# Autodesk Inventor assembly: Custom_Delta_Assembly
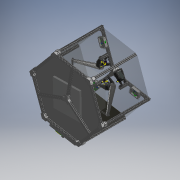
[picture p0: Inventor's stored thumbnail of the model, 180x180]
Saved by Autodesk Inventor 2019.4 (Build 234330000, 330)
## iProperties
Created: 2019-07-06
Part Number: Custom_Delta_Assembly
Document SubType Name: Assembly
Designer: Jorian Brusind
Author: Jorian Brusind
## Documents named in this file (20)
- C:\Users\Jorian Bruslind\Documents\GitHub\ECE44x_Senior_Design\Design files\Delta Robot Arm\Inventor Files\Custom_Delta\Custom_Delta_Assembly.iam
- C:\Users\Jorian Bruslind\Documents\GitHub\ECE44x_Senior_Design\Design files\Delta Robot Arm\Inventor Files\Custom_Delta\Stepper_Face.ipt
- C:\Users\Jorian Bruslind\Documents\GitHub\ECE44x_Senior_Design\Design files\Delta Robot Arm\Inventor Files\Custom_Delta\Delta_Arm.ipt
- C:\Users\Jorian Bruslind\Documents\GitHub\ECE44x_Senior_Design\Design files\Delta Robot Arm\Inventor Files\McMaster Files\5537T518_T-SLOTTED FRAMING.ipt
- C:\Users\Jorian Bruslind\Documents\GitHub\ECE44x_Senior_Design\Design files\Delta Robot Arm\Inventor Files\Custom_Delta\NEMA17_Stepper_CL42H60.ipt
- C:\Users\Jorian Bruslind\Documents\GitHub\ECE44x_Senior_Design\Design files\Delta Robot Arm\Inventor Files\Stepper_Collar\products\12196\step\model.ipt
- C:\Users\Jorian Bruslind\Documents\GitHub\ECE44x_Senior_Design\Design files\Delta Robot Arm\Inventor Files\Custom_Delta\Workarea.ipt
- C:\Users\Jorian Bruslind\Documents\GitHub\ECE44x_Senior_Design\Design files\Delta Robot Arm\Inventor Files\Custom_Delta\Frame_Skeleton.iam
- C:\Users\Jorian Bruslind\Documents\GitHub\ECE44x_Senior_Design\Design files\Delta Robot Arm\Inventor Files\Custom_Delta\350mm_2020_tslot.ipt
- C:\Users\Jorian Bruslind\Documents\GitHub\ECE44x_Senior_Design\Design files\Delta Robot Arm\Inventor Files\Custom_Delta\80_20_top_connector.ipt
- C:\Users\Jorian Bruslind\Documents\GitHub\ECE44x_Senior_Design\Design files\Delta Robot Arm\Inventor Files\McMaster Files\98861A050_LOW-STRENGTH STEEL THREADED ROD.ipt
- C:\Users\Jorian Bruslind\Documents\GitHub\ECE44x_Senior_Design\Design files\Delta Robot Arm\Inventor Files\McMaster Files\59935K140_METRIC BALL JOINT ROD END.ipt
- C:\Users\Jorian Bruslind\Documents\GitHub\ECE44x_Senior_Design\Design files\Delta Robot Arm\Inventor Files\Custom_Delta\End_Effector.iam
- C:\Users\Jorian Bruslind\Documents\GitHub\ECE44x_Senior_Design\Design files\Delta Robot Arm\Inventor Files\Custom_Delta\77mm_2020_tslot.ipt
- C:\Users\Jorian Bruslind\Documents\GitHub\ECE44x_Senior_Design\Design files\Delta Robot Arm\Inventor Files\Custom_Delta\275mm_2020_tslot.ipt
- C:\Users\Jorian Bruslind\Documents\GitHub\ECE44x_Senior_Design\Design files\Delta Robot Arm\Inventor Files\Custom_Delta\Acrylic_bottom.ipt
- C:\Users\Jorian Bruslind\Documents\GitHub\ECE44x_Senior_Design\Design files\Delta Robot Arm\Inventor Files\Custom_Delta\Motor_Node.iam
- C:\Users\Jorian Bruslind\Documents\GitHub\ECE44x_Senior_Design\Design files\Delta Robot Arm\Inventor Files\Custom_Delta\Power_Supply.ipt
- C:\Users\Jorian Bruslind\Documents\GitHub\ECE44x_Senior_Design\Design files\Delta Robot Arm\Inventor Files\Raspberry PI 3\Raspberry Pi 3.iam
- C:\Users\Jorian Bruslind\Documents\GitHub\ECE44x_Senior_Design\Design files\Delta Robot Arm\Inventor Files\Custom_Delta\Acrylic_angle_bracket.ipt
## Components (56 placed, 19 different names)
1. Stepper_Face:1 — Mate:210, Mate:211, Mate:212, Mate:216, Mate:493, Flush:5, Flush:9, Mate:506, Mate:555
2. Delta_Arm:1 — Mate:214, Mate:215, Mate:254, Mate:517, Mate:518, Mate:519, Mate:520
3. Stepper_Face:2 — Mate:222, Mate:227, Mate:230, Mate:231, Mate:491, Flush:10, Mate:505, Mate:553
4. Delta_Arm:2 — Mate:220, Mate:221, Mate:253, Mate:513, Mate:514, Mate:515, Mate:516
5. Stepper_Face:3 — Mate:217, Mate:218, Mate:226, Mate:228, Mate:495, Flush:8, Mate:507, Mate:557
6. Delta_Arm:3 — Mate:224, Mate:225, Mate:229, Mate:509, Mate:510, Mate:511, Mate:512
7. NEMA17_Stepper_CL42H60:1 — Mate:219, Mate:227, Mate:230, Mate:231
8. NEMA17_Stepper_CL42H60:2 — Mate:210, Mate:211, Mate:212, Mate:213
9. NEMA17_Stepper_CL42H60:3 — Mate:217, Mate:218, Mate:223, Mate:228
10. model:4 — Mate:223, Mate:224, Mate:225, Mate:226, Mate:229
11. model:5 — Mate:213, Mate:214, Mate:215, Mate:216, Mate:254
12. model:6 — Mate:219, Mate:220, Mate:221, Mate:222, Mate:253
13. 5537T518_T-SLOTTED FRAMING:4 — Mate:500, Mate:501, Flush:11
14. 5537T518_T-SLOTTED FRAMING:5 — Mate:496, Mate:497, Flush:13
15. 5537T518_T-SLOTTED FRAMING:6 — Mate:498, Mate:499, Flush:12
16. Workarea:1 — Flush:17, Mate:558
17. Frame_Skeleton:1 [sub-assembly] — Flush:1, Mate:490, Flush:2, Mate:492, Flush:3, Flush:4, Flush:6, Flush:7, Mate:494, Mate:496, Mate:498, Mate:500, Mate:508, Flush:11, Flush:12, Flush:13, Flush:17, Mate:559, Mate:560, Flush:18, Mate:561, Flush:19, Mate:562, Mate:563, Flush:20, Mate:564, Mate:569, Mate:570, Mate:571, Mate:573, Mate:574, Mate:576, Mate:578, Mate:581, Mate:582, Mate:587, Mate:588, Flush:26
18. 350mm_2020_tslot:1 — Flush:6, Flush:7, Mate:494, Mate:495, Flush:8, Mate:497, Mate:556, Flush:16, Mate:577, Flush:21, Flush:25
19. 350mm_2020_tslot:2 — Flush:1, Mate:490, Flush:2, Mate:491, Mate:501, Mate:502, Mate:503, Mate:504, Flush:10, Mate:552, Flush:14, Mate:579, Flush:22
20. 350mm_2020_tslot:3 — Mate:492, Flush:3, Flush:4, Mate:493, Flush:5, Flush:9, Mate:499, Mate:554, Flush:15, Mate:580, Flush:23
21. 80_20_top_connector:1 — Mate:502, Mate:503, Mate:504, Mate:505, Mate:506, Mate:507, Mate:545, Mate:558
22. 98861A050_LOW-STRENGTH STEEL THREADED ROD:1 — Mate:531, Mate:532, Mate:543, Mate:544
23. 98861A050_LOW-STRENGTH STEEL THREADED ROD:2 — Mate:529, Mate:530, Mate:541, Mate:542
24. 98861A050_LOW-STRENGTH STEEL THREADED ROD:3 — Mate:527, Mate:528, Mate:537, Mate:538
25. 98861A050_LOW-STRENGTH STEEL THREADED ROD:4 — Mate:521, Mate:522, Mate:539, Mate:540
26. 98861A050_LOW-STRENGTH STEEL THREADED ROD:5 — Mate:525, Mate:526, Mate:535, Mate:536
27. 98861A050_LOW-STRENGTH STEEL THREADED ROD:6 — Mate:523, Mate:524, Mate:533, Mate:534
28. 59935K140_METRIC BALL JOINT ROD END:1 — Mate:519, Mate:520, Mate:527, Mate:528
29. 59935K140_METRIC BALL JOINT ROD END:2 — Mate:535, Mate:536, Mate:551
30. 59935K140_METRIC BALL JOINT ROD END:3 — Mate:511, Mate:512, Mate:521, Mate:522
31. 59935K140_METRIC BALL JOINT ROD END:4 — Mate:509, Mate:510, Mate:523, Mate:524
32. 59935K140_METRIC BALL JOINT ROD END:5 — Mate:537, Mate:538, Mate:550
33. 59935K140_METRIC BALL JOINT ROD END:6 — Mate:515, Mate:516, Mate:531, Mate:532
34. 59935K140_METRIC BALL JOINT ROD END:7 — Mate:513, Mate:514, Mate:529, Mate:530
35. 59935K140_METRIC BALL JOINT ROD END:8 — Mate:543, Mate:544, Mate:546
36. 59935K140_METRIC BALL JOINT ROD END:9 — Mate:541, Mate:542, Mate:547
37. 59935K140_METRIC BALL JOINT ROD END:10 — Mate:517, Mate:518, Mate:525, Mate:526
38. 59935K140_METRIC BALL JOINT ROD END:11 — Mate:533, Mate:534, Mate:549
39. 59935K140_METRIC BALL JOINT ROD END:12 — Mate:539, Mate:540, Mate:548
40. End_Effector:1 [sub-assembly] — Mate:545, Mate:546, Mate:547, Mate:548, Mate:549, Mate:550, Mate:551
41. 77mm_2020_tslot:1 — Mate:552, Flush:14, Mate:553
42. 77mm_2020_tslot:2 — Mate:554, Flush:15, Mate:555
43. 77mm_2020_tslot:3 — Mate:556, Flush:16, Mate:557
44. 275mm_2020_tslot:1 — Mate:559, Mate:560, Flush:18, Mate:575
45. 275mm_2020_tslot:2 — Mate:561, Flush:19, Mate:562, Mate:565, Mate:566, Mate:567
46. 275mm_2020_tslot:3 — Mate:563, Flush:20, Mate:564, Mate:568, Mate:572
47. 80_20_top_connector:2 — Mate:565, Mate:566, Mate:567
48. Acrylic_bottom:1 — Mate:568, Mate:569, Mate:570
49. Acrylic_bottom:2 — Mate:571, Mate:572, Mate:573
50. Acrylic_bottom:3 — Mate:574, Mate:575, Mate:576
51. Motor_Node:1 [sub-assembly] — Mate:577, Mate:578, Flush:21
52. Motor_Node:2 [sub-assembly] — Mate:579, Mate:581, Flush:22
53. Motor_Node:3 [sub-assembly] — Mate:580, Mate:582, Flush:23
54. Power_Supply:1 — Mate:586, Flush:24, Mate:588, Flush:26
55. Raspberry Pi 3:1 [sub-assembly] — Mate:586, Flush:24
56. Acrylic_angle_bracket:1 — Mate:587, Flush:25
## Relationships (146: Mate 120, Flush 26)
- Mate:210: Stepper_Face:1 ↔ NEMA17_Stepper_CL42H60:2
- Mate:211: Stepper_Face:1 ↔ NEMA17_Stepper_CL42H60:2
- Mate:212: Stepper_Face:1 ↔ NEMA17_Stepper_CL42H60:2
- Mate:213: NEMA17_Stepper_CL42H60:2 ↔ model:5
- Mate:214: Delta_Arm:1 ↔ model:5
- Mate:215: Delta_Arm:1 ↔ model:5
- Mate:216: Stepper_Face:1 ↔ model:5
- Mate:217: Stepper_Face:3 ↔ NEMA17_Stepper_CL42H60:3
- Mate:218: Stepper_Face:3 ↔ NEMA17_Stepper_CL42H60:3
- Mate:219: NEMA17_Stepper_CL42H60:1 ↔ model:6
- Mate:220: Delta_Arm:2 ↔ model:6
- Mate:221: Delta_Arm:2 ↔ model:6
- Mate:222: Stepper_Face:2 ↔ model:6
- Mate:223: NEMA17_Stepper_CL42H60:3 ↔ model:4
- Mate:224: Delta_Arm:3 ↔ model:4
- Mate:225: Delta_Arm:3 ↔ model:4
- Mate:226: Stepper_Face:3 ↔ model:4
- Mate:227: Stepper_Face:2 ↔ NEMA17_Stepper_CL42H60:1
- Mate:228: Stepper_Face:3 ↔ NEMA17_Stepper_CL42H60:3
- Mate:229: Delta_Arm:3 ↔ model:4
- Mate:230: Stepper_Face:2 ↔ NEMA17_Stepper_CL42H60:1
- Mate:231: Stepper_Face:2 ↔ NEMA17_Stepper_CL42H60:1
- Mate:253: Delta_Arm:2 ↔ model:6
- Mate:254: Delta_Arm:1 ↔ model:5
- Flush:1: Frame_Skeleton:1 ↔ 350mm_2020_tslot:2
- Mate:490: Frame_Skeleton:1 ↔ 350mm_2020_tslot:2
- Flush:2: Frame_Skeleton:1 ↔ 350mm_2020_tslot:2
- Mate:491: Stepper_Face:2 ↔ 350mm_2020_tslot:2
- Mate:492: Frame_Skeleton:1 ↔ 350mm_2020_tslot:3
- Flush:3: Frame_Skeleton:1 ↔ 350mm_2020_tslot:3
- Flush:4: Frame_Skeleton:1 ↔ 350mm_2020_tslot:3
- Mate:493: Stepper_Face:1 ↔ 350mm_2020_tslot:3
- Flush:5: Stepper_Face:1 ↔ 350mm_2020_tslot:3
- Flush:6: Frame_Skeleton:1 ↔ 350mm_2020_tslot:1
- Flush:7: Frame_Skeleton:1 ↔ 350mm_2020_tslot:1
- Mate:494: Frame_Skeleton:1 ↔ 350mm_2020_tslot:1
- Mate:495: Stepper_Face:3 ↔ 350mm_2020_tslot:1
- Flush:8: Stepper_Face:3 ↔ 350mm_2020_tslot:1
- Flush:9: Stepper_Face:1 ↔ 350mm_2020_tslot:3
- Mate:496: 5537T518_T-SLOTTED FRAMING:5 ↔ Frame_Skeleton:1
- Mate:497: 5537T518_T-SLOTTED FRAMING:5 ↔ 350mm_2020_tslot:1
- Mate:498: 5537T518_T-SLOTTED FRAMING:6 ↔ Frame_Skeleton:1
- Mate:499: 5537T518_T-SLOTTED FRAMING:6 ↔ 350mm_2020_tslot:3
- Mate:500: 5537T518_T-SLOTTED FRAMING:4 ↔ Frame_Skeleton:1
- Mate:501: 5537T518_T-SLOTTED FRAMING:4 ↔ 350mm_2020_tslot:2
- Mate:502: 350mm_2020_tslot:2 ↔ 80_20_top_connector:1
- Mate:503 (0.5 mm): 350mm_2020_tslot:2 ↔ 80_20_top_connector:1
- Mate:504 (0.5 mm): 350mm_2020_tslot:2 ↔ 80_20_top_connector:1
- Flush:10: Stepper_Face:2 ↔ 350mm_2020_tslot:2
- Mate:505 (120 mm): Stepper_Face:2 ↔ 80_20_top_connector:1
- Mate:506 (120 mm): Stepper_Face:1 ↔ 80_20_top_connector:1
- Mate:507 (120 mm): Stepper_Face:3 ↔ 80_20_top_connector:1
- Mate:508: Frame_Skeleton:1
- Flush:11: 5537T518_T-SLOTTED FRAMING:4 ↔ Frame_Skeleton:1
- Flush:12: 5537T518_T-SLOTTED FRAMING:6 ↔ Frame_Skeleton:1
- Flush:13: 5537T518_T-SLOTTED FRAMING:5 ↔ Frame_Skeleton:1
- Mate:509: Delta_Arm:3 ↔ 59935K140_METRIC BALL JOINT ROD END:4
- Mate:510 (10 mm): Delta_Arm:3 ↔ 59935K140_METRIC BALL JOINT ROD END:4
- Mate:511: Delta_Arm:3 ↔ 59935K140_METRIC BALL JOINT ROD END:3
- Mate:512 (10 mm): Delta_Arm:3 ↔ 59935K140_METRIC BALL JOINT ROD END:3
- Mate:513: Delta_Arm:2 ↔ 59935K140_METRIC BALL JOINT ROD END:7
- Mate:514 (10 mm): Delta_Arm:2 ↔ 59935K140_METRIC BALL JOINT ROD END:7
- Mate:515: Delta_Arm:2 ↔ 59935K140_METRIC BALL JOINT ROD END:6
- Mate:516 (10 mm): Delta_Arm:2 ↔ 59935K140_METRIC BALL JOINT ROD END:6
- Mate:517: Delta_Arm:1 ↔ 59935K140_METRIC BALL JOINT ROD END:10
- Mate:518 (10 mm): Delta_Arm:1 ↔ 59935K140_METRIC BALL JOINT ROD END:10
- Mate:519: Delta_Arm:1 ↔ 59935K140_METRIC BALL JOINT ROD END:1
- Mate:520 (10 mm): Delta_Arm:1 ↔ 59935K140_METRIC BALL JOINT ROD END:1
- Mate:521: 98861A050_LOW-STRENGTH STEEL THREADED ROD:4 ↔ 59935K140_METRIC BALL JOINT ROD END:3
- Mate:522: 98861A050_LOW-STRENGTH STEEL THREADED ROD:4 ↔ 59935K140_METRIC BALL JOINT ROD END:3
- Mate:523: 98861A050_LOW-STRENGTH STEEL THREADED ROD:6 ↔ 59935K140_METRIC BALL JOINT ROD END:4
- Mate:524: 98861A050_LOW-STRENGTH STEEL THREADED ROD:6 ↔ 59935K140_METRIC BALL JOINT ROD END:4
- Mate:525: 98861A050_LOW-STRENGTH STEEL THREADED ROD:5 ↔ 59935K140_METRIC BALL JOINT ROD END:10
- Mate:526: 98861A050_LOW-STRENGTH STEEL THREADED ROD:5 ↔ 59935K140_METRIC BALL JOINT ROD END:10
- Mate:527: 98861A050_LOW-STRENGTH STEEL THREADED ROD:3 ↔ 59935K140_METRIC BALL JOINT ROD END:1
- Mate:528: 98861A050_LOW-STRENGTH STEEL THREADED ROD:3 ↔ 59935K140_METRIC BALL JOINT ROD END:1
- Mate:529: 98861A050_LOW-STRENGTH STEEL THREADED ROD:2 ↔ 59935K140_METRIC BALL JOINT ROD END:7
- Mate:530: 98861A050_LOW-STRENGTH STEEL THREADED ROD:2 ↔ 59935K140_METRIC BALL JOINT ROD END:7
- Mate:531: 98861A050_LOW-STRENGTH STEEL THREADED ROD:1 ↔ 59935K140_METRIC BALL JOINT ROD END:6
- Mate:532: 98861A050_LOW-STRENGTH STEEL THREADED ROD:1 ↔ 59935K140_METRIC BALL JOINT ROD END:6
- Mate:533: 98861A050_LOW-STRENGTH STEEL THREADED ROD:6 ↔ 59935K140_METRIC BALL JOINT ROD END:11
- Mate:534 (-10 mm): 98861A050_LOW-STRENGTH STEEL THREADED ROD:6 ↔ 59935K140_METRIC BALL JOINT ROD END:11
- Mate:535: 98861A050_LOW-STRENGTH STEEL THREADED ROD:5 ↔ 59935K140_METRIC BALL JOINT ROD END:2
- Mate:536 (-10 mm): 98861A050_LOW-STRENGTH STEEL THREADED ROD:5 ↔ 59935K140_METRIC BALL JOINT ROD END:2
- Mate:537: 98861A050_LOW-STRENGTH STEEL THREADED ROD:3 ↔ 59935K140_METRIC BALL JOINT ROD END:5
- Mate:538 (-10 mm): 98861A050_LOW-STRENGTH STEEL THREADED ROD:3 ↔ 59935K140_METRIC BALL JOINT ROD END:5
- Mate:539: 98861A050_LOW-STRENGTH STEEL THREADED ROD:4 ↔ 59935K140_METRIC BALL JOINT ROD END:12
- Mate:540 (-10 mm): 98861A050_LOW-STRENGTH STEEL THREADED ROD:4 ↔ 59935K140_METRIC BALL JOINT ROD END:12
- Mate:541: 98861A050_LOW-STRENGTH STEEL THREADED ROD:2 ↔ 59935K140_METRIC BALL JOINT ROD END:9
- Mate:542 (-10 mm): 98861A050_LOW-STRENGTH STEEL THREADED ROD:2 ↔ 59935K140_METRIC BALL JOINT ROD END:9
- Mate:543: 98861A050_LOW-STRENGTH STEEL THREADED ROD:1 ↔ 59935K140_METRIC BALL JOINT ROD END:8
- Mate:544 (-10 mm): 98861A050_LOW-STRENGTH STEEL THREADED ROD:1 ↔ 59935K140_METRIC BALL JOINT ROD END:8
- Mate:545: 80_20_top_connector:1 ↔ End_Effector:1
- Mate:546: 59935K140_METRIC BALL JOINT ROD END:8 ↔ End_Effector:1
- Mate:547: 59935K140_METRIC BALL JOINT ROD END:9 ↔ End_Effector:1
- Mate:548: 59935K140_METRIC BALL JOINT ROD END:12 ↔ End_Effector:1
- Mate:549: 59935K140_METRIC BALL JOINT ROD END:11 ↔ End_Effector:1
- Mate:550: 59935K140_METRIC BALL JOINT ROD END:5 ↔ End_Effector:1
- Mate:551: 59935K140_METRIC BALL JOINT ROD END:2 ↔ End_Effector:1
- Mate:552: 350mm_2020_tslot:2 ↔ 77mm_2020_tslot:1
- Flush:14: 350mm_2020_tslot:2 ↔ 77mm_2020_tslot:1
- Mate:553: Stepper_Face:2 ↔ 77mm_2020_tslot:1
- Mate:554: 350mm_2020_tslot:3 ↔ 77mm_2020_tslot:2
- Flush:15: 350mm_2020_tslot:3 ↔ 77mm_2020_tslot:2
- Mate:555: Stepper_Face:1 ↔ 77mm_2020_tslot:2
- Mate:556: 350mm_2020_tslot:1 ↔ 77mm_2020_tslot:3
- Flush:16: 350mm_2020_tslot:1 ↔ 77mm_2020_tslot:3
- Mate:557: Stepper_Face:3 ↔ 77mm_2020_tslot:3
- Flush:17: Workarea:1 ↔ Frame_Skeleton:1
- Mate:558: Workarea:1 ↔ 80_20_top_connector:1
- Mate:559: Frame_Skeleton:1 ↔ 275mm_2020_tslot:1
- Mate:560 (140.5 mm): Frame_Skeleton:1 ↔ 275mm_2020_tslot:1
- Flush:18: Frame_Skeleton:1 ↔ 275mm_2020_tslot:1
- Mate:561: Frame_Skeleton:1 ↔ 275mm_2020_tslot:2
- Flush:19: Frame_Skeleton:1 ↔ 275mm_2020_tslot:2
- Mate:562 (140.5 mm): Frame_Skeleton:1 ↔ 275mm_2020_tslot:2
- Mate:563: Frame_Skeleton:1 ↔ 275mm_2020_tslot:3
- Flush:20: Frame_Skeleton:1 ↔ 275mm_2020_tslot:3
- Mate:564 (140.5 mm): Frame_Skeleton:1 ↔ 275mm_2020_tslot:3
- Mate:565: 275mm_2020_tslot:2 ↔ 80_20_top_connector:2
- Mate:566 (0.5 mm): 275mm_2020_tslot:2 ↔ 80_20_top_connector:2
- Mate:567 (0.5 mm): 275mm_2020_tslot:2 ↔ 80_20_top_connector:2
- Mate:568: 275mm_2020_tslot:3 ↔ Acrylic_bottom:1
- Mate:569: Frame_Skeleton:1 ↔ Acrylic_bottom:1
- Mate:570: Frame_Skeleton:1 ↔ Acrylic_bottom:1
- Mate:571: Frame_Skeleton:1 ↔ Acrylic_bottom:2
- Mate:572: 275mm_2020_tslot:3 ↔ Acrylic_bottom:2
- Mate:573: Frame_Skeleton:1 ↔ Acrylic_bottom:2
- Mate:574: Frame_Skeleton:1 ↔ Acrylic_bottom:3
- Mate:575: 275mm_2020_tslot:1 ↔ Acrylic_bottom:3
- Mate:576: Frame_Skeleton:1 ↔ Acrylic_bottom:3
- Mate:577: 350mm_2020_tslot:1 ↔ Motor_Node:1
- Mate:578 (60 mm): Frame_Skeleton:1 ↔ Motor_Node:1
- Flush:21 (-20 mm): 350mm_2020_tslot:1 ↔ Motor_Node:1
- Mate:579: 350mm_2020_tslot:2 ↔ Motor_Node:2
- Mate:580: 350mm_2020_tslot:3 ↔ Motor_Node:3
- Mate:581 (60 mm): Frame_Skeleton:1 ↔ Motor_Node:2
- Flush:22 (-20 mm): 350mm_2020_tslot:2 ↔ Motor_Node:2
- Mate:582 (60 mm): Frame_Skeleton:1 ↔ Motor_Node:3
- Flush:23 (-20 mm): 350mm_2020_tslot:3 ↔ Motor_Node:3
- Mate:586: Power_Supply:1 ↔ Raspberry Pi 3:1
- Flush:24: Power_Supply:1 ↔ Raspberry Pi 3:1
- Mate:587: Frame_Skeleton:1 ↔ Acrylic_angle_bracket:1
- Flush:25 (50 mm): 350mm_2020_tslot:1 ↔ Acrylic_angle_bracket:1
- Mate:588: Frame_Skeleton:1 ↔ Power_Supply:1
- Flush:26 (30 mm): Frame_Skeleton:1 ↔ Power_Supply:1
